# Autodesk Inventor assembly: Assieme2
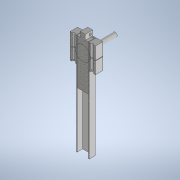
[picture p0: Inventor's stored thumbnail of the model, 180x180]
Saved by Autodesk Inventor 2020 (Build 240168000, 168)
## iProperties
Created: 2019-10-11
Part Number: Assieme2
Document SubType Name: Assembly
Designer: socci
Author: socci
## Documents named in this file (5)
- C:\Users\socci\Desktop\mv-Project\04_PartDraw\Modello_3D.iam
- C:\Users\socci\Desktop\mv-Project\04_PartDraw\Componenti\1_Asse_cuscinetti.ipt
- C:\Users\socci\Desktop\mv-Project\04_PartDraw\Componenti\2_Connettore_inf_sup.ipt
- C:\Users\socci\Desktop\mv-Project\04_PartDraw\Componenti\3_Connettore_inf_INF.ipt
- C:\Users\socci\Desktop\mv-Project\04_PartDraw\Componenti\4_barra.ipt
## Components (4 placed, 4 different names)
1. 1_Asse_cuscinetti:1 — Inserimento:1, Inserimento:2
2. 2_Connettore_inf_sup:1 — Inserimento:1, Coincidente:1, Coincidente:2
3. 3_Connettore_inf_INF:1 — Inserimento:2
4. 4_barra:1 — Coincidente:1, Coincidente:2
## Relationships (4: Insert 2, Mate 2)
- Inserimento:1: 1_Asse_cuscinetti:1 ↔ 2_Connettore_inf_sup:1
- Inserimento:2: 1_Asse_cuscinetti:1 ↔ 3_Connettore_inf_INF:1
- Coincidente:1 [Mate]: 2_Connettore_inf_sup:1 ↔ 4_barra:1
- Coincidente:2 [Mate]: 2_Connettore_inf_sup:1 ↔ 4_barra:1
